# Autodesk Inventor assembly: Zalepka_osi_Z
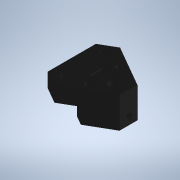
[picture p0: Inventor's stored thumbnail of the model, 180x180]
Saved by Autodesk Inventor 2021 (Build 250183000, 183)
## iProperties
Created: 2021-07-30
Part Number: Zalepka_osi_Z
Document SubType Name: Assembly
Designer: Janusz
Author: Janusz
Revision Number: ANY
## Documents named in this file (2)
- D:\ROBOT\Zalepka_osi_Z.iam
- D:\ROBOT\Zalepka_osi_Z_cz_1Zlo_Podstawa pod chwytak.ipt
## Components (1 placed, 1 different names)
1. Zalepka_osi_Z_cz_1Zlo_Podstawa pod chwytak_26 — Zestawiające:1
## Relationships (1: Mate 1)
- Zestawiające:1 [Mate]: Zalepka_osi_Z_cz_1Zlo_Podstawa pod chwytak_26
